# Autodesk Inventor assembly: FINAL
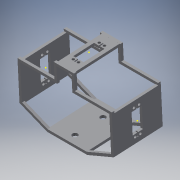
[picture p0: Inventor's stored thumbnail of the model, 180x180]
Saved by Autodesk Inventor 2018 (Build 220112000, 112)
## iProperties
Created: 2018-04-02
Part Number: FINAL
Document SubType Name: Assembly
Designer: Lilia
Author: Lilia
## Documents named in this file (5)
- C:\Users\Public\Documents\Autodesk\.desktop-connect\.docstore\guided-tutorial-plugin\INVNTOR\2018\ENU\455171510111540556\TutorialModelPath\FINAL.iam
- C:\Users\Public\Documents\Autodesk\.desktop-connect\.docstore\guided-tutorial-plugin\INVNTOR\2018\ENU\455171510111540556\TutorialModelPath\Buste Epaule.ipt
- C:\Users\Public\Documents\Autodesk\.desktop-connect\.docstore\guided-tutorial-plugin\INVNTOR\2018\ENU\455171510111540556\TutorialModelPath\Buste1.ipt
- C:\Users\Public\Documents\Autodesk\.desktop-connect\.docstore\guided-tutorial-plugin\INVNTOR\2018\ENU\455171510111540556\TutorialModelPath\Cou-3.ipt
- C:\Users\Public\Documents\Autodesk\.desktop-connect\.docstore\guided-tutorial-plugin\INVNTOR\2018\ENU\455171510111540556\TutorialModelPath\Buste3-2.ipt
## Components (6 placed, 4 different names)
1. Buste Epaule:1 — Mate:1, Mate:5, Mate:12
2. Buste1:1 — Mate:1, Mate:2, Mate:10, Mate:11, Mate:12, Mate:13
3. Buste Epaule:2 — Mate:2, Mate:6
4. Cou-3:1 — Mate:13
5. Buste1:2 — Mate:5, Mate:6
6. Buste3-2:1 — Mate:10, Mate:11
## Relationships (8: Mate 8)
- Mate:1: Buste Epaule:1 ↔ Buste1:1
- Mate:2: Buste1:1 ↔ Buste Epaule:2
- Mate:5: Buste Epaule:1 ↔ Buste1:2
- Mate:6: Buste Epaule:2 ↔ Buste1:2
- Mate:10: Buste1:1 ↔ Buste3-2:1
- Mate:11: Buste1:1 ↔ Buste3-2:1
- Mate:12: Buste Epaule:1 ↔ Buste1:1
- Mate:13: Buste1:1 ↔ Cou-3:1
